# Autodesk Inventor assembly: Claw
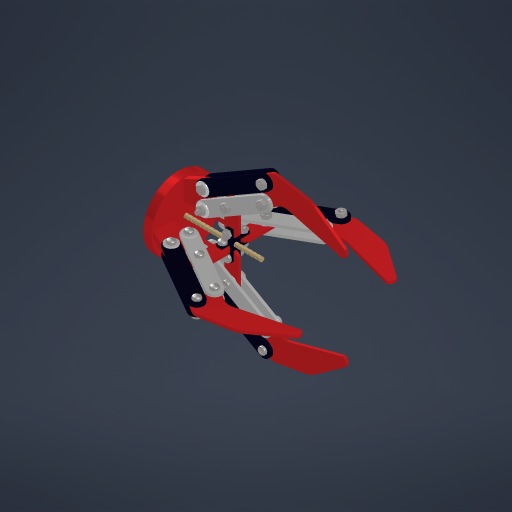
[picture p0: Inventor's stored thumbnail of the model, 512x512]
Saved by Autodesk Inventor 2023 (Build 270158000, 158)
## iProperties
Created: 2023-04-10
Part Number: Claw
Document SubType Name: Assembly
Designer: vatdu
Author: vatdu
## Documents named in this file (16)
- C:\Users\vatdu\Desktop\CRYSTAL MARK II\Arm\Claw\Claw.iam
- C:\Users\vatdu\Desktop\CRYSTAL MARK II\Components\DVD Stepper Motor\Stepper motor CD Drive.iam
- C:\Users\vatdu\Desktop\CRYSTAL MARK II\Arm\Claw\Base.ipt
- C:\Users\vatdu\Desktop\CRYSTAL MARK II\Arm\Claw\Side support 1.ipt
- C:\Users\vatdu\Documents\Inventor\Content Center Files\R2023\en-US\BS EN ISO 7045 H\EN ISO 7045 - M3 x 12 - 4.8 - H(1).ipt
- C:\Users\vatdu\Documents\Inventor\Content Center Files\R2023\en-US\AS 1474(1)\AS 1474 - M3(1).ipt
- C:\Users\vatdu\Documents\Inventor\Content Center Files\R2023\en-US\AS 1237 (3.1)\AS 1237 - 4 mm(1)Aluminium-6061.ipt
- C:\Users\vatdu\Desktop\CRYSTAL MARK II\Arm\Claw\Side Support 2.ipt
- C:\Users\vatdu\Documents\Inventor\Content Center Files\R2023\en-US\BS EN ISO 7045 H\EN ISO 7045 - M3 x 14 - 4.8 - H(1).ipt
- C:\Users\vatdu\Desktop\CRYSTAL MARK II\Arm\Claw\Middle support.ipt
- C:\Users\vatdu\Desktop\CRYSTAL MARK II\Arm\Claw\Center Connector.ipt
- C:\Users\vatdu\Documents\Inventor\Content Center Files\R2023\en-US\BS EN ISO 7045 H\EN ISO 7045 - M3 x 10 - 4.8 - H(1).ipt
- C:\Users\vatdu\Documents\Inventor\Content Center Files\R2023\en-US\AS 1474(1)\AS 1474 - M2.5(1).ipt
- C:\Users\vatdu\Desktop\CRYSTAL MARK II\Arm\Claw\Claw Tip.ipt
- C:\Users\vatdu\Documents\Inventor\Content Center Files\R2023\en-US\AS 1237 (2.1)\AS 1237 - 3.ipt
- C:\Users\vatdu\Documents\Inventor\Content Center Files\R2023\en-US\ANSI B18.2.4.2M\ANSI B18.2.4.2M - M3x0.5 - 5.5.ipt
## Components (124 placed, 15 different names)
1. Stepper motor CD Drive:1 [sub-assembly] — Rotational:1, Rotational:19
2. Base:1 — Rotational:1, Rotational:2, Rotational:3, Rotational:8, Rotational:9
3. AS 1474 - Metric M3:10 — Rotational:18
4. Center Connector:1 — Rotational:19, Rotational:20, Insert:1
5. AS 1237 (2.1) 3:2 — Insert:3
6. AS 1237 (2.1) 3:4 — Insert:5
7. AS 1237 (2.1) 3:5 — Insert:6
8. AS 1237 (2.1) 3:7 — Insert:8
9. AS 1237 (2.1) 3:9 — Insert:10
10. AS 1237 (2.1) 3:10 — Insert:11
11. ANSI B18.2.4.2M M3x0.5:2 — Insert:13
12. ANSI B18.2.4.2M M3x0.5:4 — Insert:15
13. BS EN ISO 7045 H - Metric M3 x 12 - 4.8 - H:1 — Rotational:5
14. AS 1237 (3.1) 4 mm - Aluminum 6061:1 — Rotational:4, Rotational:5
15. Side support 1:2 — Rotational:3, Rotational:4
16. Side support 1:1 — Rotational:2, Rotational:6
17. AS 1474 - Metric M3:1 — Rotational:7
18. AS 1237 (3.1) 4 mm - Aluminum 6061:2 — Rotational:6, Rotational:7
19. BS EN ISO 7045 H - Metric M3 x 12 - 4.8 - H:2
20. AS 1237 (3.1) 4 mm - Aluminum 6061:3
21. Side support 1:3
22. Side support 1:4
23. AS 1474 - Metric M3:2
24. AS 1237 (3.1) 4 mm - Aluminum 6061:4
25. BS EN ISO 7045 H - Metric M3 x 12 - 4.8 - H:3
26. AS 1237 (3.1) 4 mm - Aluminum 6061:5
27. Side support 1:5 — Insert:7, Insert:8, Rotational:23
28. Side support 1:6 — Insert:2, Insert:3, Insert:12, Insert:13
29. AS 1474 - Metric M3:3
30. AS 1237 (3.1) 4 mm - Aluminum 6061:6
31. BS EN ISO 7045 H - Metric M3 x 12 - 4.8 - H:4
32. AS 1237 (3.1) 4 mm - Aluminum 6061:7
33. Side support 1:7
34. Side support 1:8
35. AS 1474 - Metric M3:4
36. AS 1237 (3.1) 4 mm - Aluminum 6061:8
37. Side Support 2:2 — Rotational:9, Rotational:11
38. AS 1474 - Metric M3:6 — Rotational:13
39. AS 1237 (3.1) 4 mm - Aluminum 6061:9 — Rotational:11, Rotational:13
40. Side Support 2:1 — Rotational:8, Rotational:10
41. AS 1237 (3.1) 4 mm - Aluminum 6061:10 — Rotational:10, Rotational:12
42. BS EN ISO 7045 H - Metric M3 x 14 - 4.8 - H:1 — Rotational:12
43. Side Support 2:3 — Rotational:15, Rotational:18, Insert:4, Insert:5, Insert:6, Insert:14, Insert:15, Insert:16
44. AS 1474 - Metric M3:7
45. AS 1237 (3.1) 4 mm - Aluminum 6061:11
46. Side Support 2:4 — Rotational:14, Rotational:17, Insert:9, Insert:10, Insert:11, Rotational:22
47. AS 1237 (3.1) 4 mm - Aluminum 6061:12
48. BS EN ISO 7045 H - Metric M3 x 14 - 4.8 - H:2
49. Side Support 2:5
50. AS 1474 - Metric M3:8
51. AS 1237 (3.1) 4 mm - Aluminum 6061:13
52. Side Support 2:6
53. AS 1237 (3.1) 4 mm - Aluminum 6061:14
54. BS EN ISO 7045 H - Metric M3 x 14 - 4.8 - H:3
55. Side Support 2:7
56. AS 1474 - Metric M3:9
57. AS 1237 (3.1) 4 mm - Aluminum 6061:15
58. Side Support 2:8
59. AS 1237 (3.1) 4 mm - Aluminum 6061:16
60. BS EN ISO 7045 H - Metric M3 x 14 - 4.8 - H:4
61. BS EN ISO 7045 H - Metric M3 x 12 - 4.8 - H:6 — Rotational:22
62. BS EN ISO 7045 H - Metric M3 x 12 - 4.8 - H:7 — Rotational:23
63. Claw Tip:1 — Rotational:21
64. BS EN ISO 7045 H - Metric M3 x 12 - 4.8 - H:5 — Rotational:17
65. BS EN ISO 7045 H - Metric M3 x 10 - 4.8 - H:1 — Rotational:20
66. Middle support:1 — Rotational:16
67. AS 1237 (3.1) 4 mm - Aluminum 6061:18 — Rotational:14
68. AS 1237 (3.1) 4 mm - Aluminum 6061:17 — Rotational:15, Rotational:16
69. ANSI B18.2.4.2M M3x0.5:5 — Insert:16
70. AS 1474 - Metric M2.5:1 — Insert:1
71. ANSI B18.2.4.2M M3x0.5:3 — Insert:14
72. ANSI B18.2.4.2M M3x0.5:1 — Insert:12
73. AS 1237 (2.1) 3:8 — Insert:9
74. AS 1237 (2.1) 3:3 — Insert:4, Rotational:21
75. AS 1237 (2.1) 3:1 — Insert:2
76. AS 1237 (2.1) 3:6 — Insert:7
77. BS EN ISO 7045 H - Metric M3 x 12 - 4.8 - H:8
78. BS EN ISO 7045 H - Metric M3 x 12 - 4.8 - H:9
79. Claw Tip:2
80. BS EN ISO 7045 H - Metric M3 x 12 - 4.8 - H:10
81. BS EN ISO 7045 H - Metric M3 x 10 - 4.8 - H:2
82. Middle support:2
83. AS 1237 (3.1) 4 mm - Aluminum 6061:19
84. AS 1237 (3.1) 4 mm - Aluminum 6061:20
85. ANSI B18.2.4.2M M3x0.5:6
86. AS 1474 - Metric M2.5:2
87. ANSI B18.2.4.2M M3x0.5:7
88. ANSI B18.2.4.2M M3x0.5:8
89. AS 1237 (2.1) 3:11
90. AS 1237 (2.1) 3:12
91. AS 1237 (2.1) 3:13
92. AS 1237 (2.1) 3:14
93. BS EN ISO 7045 H - Metric M3 x 12 - 4.8 - H:11
94. BS EN ISO 7045 H - Metric M3 x 12 - 4.8 - H:12
95. Claw Tip:3
96. BS EN ISO 7045 H - Metric M3 x 12 - 4.8 - H:13
97. BS EN ISO 7045 H - Metric M3 x 10 - 4.8 - H:3
98. Middle support:3
99. AS 1237 (3.1) 4 mm - Aluminum 6061:21
100. AS 1237 (3.1) 4 mm - Aluminum 6061:22
101. ANSI B18.2.4.2M M3x0.5:9
102. AS 1474 - Metric M2.5:3
103. ANSI B18.2.4.2M M3x0.5:10
104. ANSI B18.2.4.2M M3x0.5:11
105. AS 1237 (2.1) 3:15
106. AS 1237 (2.1) 3:16
107. AS 1237 (2.1) 3:17
108. AS 1237 (2.1) 3:18
109. BS EN ISO 7045 H - Metric M3 x 12 - 4.8 - H:14
110. BS EN ISO 7045 H - Metric M3 x 12 - 4.8 - H:15
111. Claw Tip:4
112. BS EN ISO 7045 H - Metric M3 x 12 - 4.8 - H:16
113. BS EN ISO 7045 H - Metric M3 x 10 - 4.8 - H:4
114. Middle support:4
115. AS 1237 (3.1) 4 mm - Aluminum 6061:23
116. AS 1237 (3.1) 4 mm - Aluminum 6061:24
117. ANSI B18.2.4.2M M3x0.5:12
118. AS 1474 - Metric M2.5:4
119. ANSI B18.2.4.2M M3x0.5:13
120. ANSI B18.2.4.2M M3x0.5:14
121. AS 1237 (2.1) 3:19
122. AS 1237 (2.1) 3:20
123. AS 1237 (2.1) 3:21
124. AS 1237 (2.1) 3:22
## Component patterns: (4 elements, first: BS EN ISO 7045 H - Metric M3 x 12 - 4.8 - H:1 + AS 1237 (3.1) 4 mm - Aluminum 6061:1 + Side support 1:2 + Side support 1:1 + AS 1474 - Metric M3:1 + AS 1237 (3.1) 4 mm - Aluminum 6061:2), (4 elements, first: Side Support 2:2 + AS 1474 - Metric M3:6 + AS 1237 (3.1) 4 mm - Aluminum 6061:9 + Side Support 2:1 + AS 1237 (3.1) 4 mm - Aluminum 6061:10 + BS EN ISO 7045 H - Metric M3 x 14 - 4.8 - H:1), (4 elements, first: BS EN ISO 7045 H - Metric M3 x 12 - 4.8 - H:6 + BS EN ISO 7045 H - Metric M3 x 12 - 4.8 - H:7 + Claw Tip:1 + BS EN ISO 7045 H - Metric M3 x 12 - 4.8 - H:5 + BS EN ISO 7045 H - Metric M3 x 10 - 4.8 - H:1 + Middle support:1 + AS 1237 (3.1) 4 mm - Aluminum 6061:18 + AS 1237 (3.1) 4 mm - Aluminum 6061:17 + ANSI B18.2.4.2M M3x0.5:5 + AS 1474 - Metric M2.5:1 + ANSI B18.2.4.2M M3x0.5:3 + ANSI B18.2.4.2M M3x0.5:1 + AS 1237 (2.1) 3:8 + AS 1237 (2.1) 3:3 + AS 1237 (2.1) 3:1 + AS 1237 (2.1) 3:6)
## Relationships (39: RevoluteJoint 23, Insert 16)
- Rotational:1 [RevoluteJoint]: Stepper motor CD Drive:1 ↔ Base:1
- Rotational:2 [RevoluteJoint]: Base:1 ↔ Side support 1:1
- Rotational:3 [RevoluteJoint]: Base:1 ↔ Side support 1:2
- Rotational:4 [RevoluteJoint]: AS 1237 (3.1) 4 mm - Aluminum 6061:1 ↔ Side support 1:2
- Rotational:5 [RevoluteJoint]: BS EN ISO 7045 H - Metric M3 x 12 - 4.8 - H:1 ↔ AS 1237 (3.1) 4 mm - Aluminum 6061:1
- Rotational:6 [RevoluteJoint]: Side support 1:1 ↔ AS 1237 (3.1) 4 mm - Aluminum 6061:2
- Rotational:7 [RevoluteJoint]: AS 1474 - Metric M3:1 ↔ AS 1237 (3.1) 4 mm - Aluminum 6061:2
- Rotational:8 [RevoluteJoint]: Base:1 ↔ Side Support 2:1
- Rotational:9 [RevoluteJoint]: Base:1 ↔ Side Support 2:2
- Rotational:10 [RevoluteJoint]: Side Support 2:1 ↔ AS 1237 (3.1) 4 mm - Aluminum 6061:10
- Rotational:11 [RevoluteJoint]: Side Support 2:2 ↔ AS 1237 (3.1) 4 mm - Aluminum 6061:9
- Rotational:12 [RevoluteJoint]: AS 1237 (3.1) 4 mm - Aluminum 6061:10 ↔ BS EN ISO 7045 H - Metric M3 x 14 - 4.8 - H:1
- Rotational:13 [RevoluteJoint]: AS 1474 - Metric M3:6 ↔ AS 1237 (3.1) 4 mm - Aluminum 6061:9
- Rotational:14 [RevoluteJoint]: Side Support 2:4 ↔ AS 1237 (3.1) 4 mm - Aluminum 6061:18
- Rotational:15 [RevoluteJoint]: Side Support 2:3 ↔ AS 1237 (3.1) 4 mm - Aluminum 6061:17
- Rotational:16 [RevoluteJoint] (-0.19 mm): Middle support:1 ↔ AS 1237 (3.1) 4 mm - Aluminum 6061:17
- Rotational:17 [RevoluteJoint]: Side Support 2:4 ↔ BS EN ISO 7045 H - Metric M3 x 12 - 4.8 - H:5
- Rotational:18 [RevoluteJoint]: AS 1474 - Metric M3:10 ↔ Side Support 2:3
- Rotational:19 [RevoluteJoint] (19 mm): Stepper motor CD Drive:1 ↔ Center Connector:1
- Rotational:20 [RevoluteJoint]: Center Connector:1 ↔ BS EN ISO 7045 H - Metric M3 x 10 - 4.8 - H:1
- Insert:1: Center Connector:1 ↔ AS 1474 - Metric M2.5:1
- Insert:2: Side support 1:6 ↔ AS 1237 (2.1) 3:1
- Insert:3: AS 1237 (2.1) 3:2 ↔ Side support 1:6
- Insert:4: Side Support 2:3 ↔ AS 1237 (2.1) 3:3
- Insert:5: AS 1237 (2.1) 3:4 ↔ Side Support 2:3
- Insert:6: AS 1237 (2.1) 3:5 ↔ Side Support 2:3
- Insert:7: Side support 1:5 ↔ AS 1237 (2.1) 3:6
- Insert:8: AS 1237 (2.1) 3:7 ↔ Side support 1:5
- Insert:9: Side Support 2:4 ↔ AS 1237 (2.1) 3:8
- Insert:10: AS 1237 (2.1) 3:9 ↔ Side Support 2:4
- Insert:11: AS 1237 (2.1) 3:10 ↔ Side Support 2:4
- Rotational:21 [RevoluteJoint] (-0.5 mm): Claw Tip:1 ↔ AS 1237 (2.1) 3:3
- Rotational:22 [RevoluteJoint]: Side Support 2:4 ↔ BS EN ISO 7045 H - Metric M3 x 12 - 4.8 - H:6
- Rotational:23 [RevoluteJoint]: Side support 1:5 ↔ BS EN ISO 7045 H - Metric M3 x 12 - 4.8 - H:7
- Insert:12: Side support 1:6 ↔ ANSI B18.2.4.2M M3x0.5:1
- Insert:13: ANSI B18.2.4.2M M3x0.5:2 ↔ Side support 1:6
- Insert:14: Side Support 2:3 ↔ ANSI B18.2.4.2M M3x0.5:3
- Insert:15: ANSI B18.2.4.2M M3x0.5:4 ↔ Side Support 2:3
- Insert:16: Side Support 2:3 ↔ ANSI B18.2.4.2M M3x0.5:5
